# Autodesk Inventor assembly: final
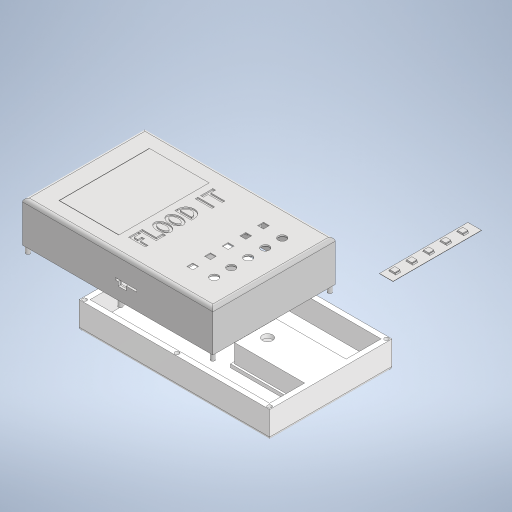
[picture p0: Inventor's stored thumbnail of the model, 512x512]
Saved by Autodesk Inventor 2023 (Build 270158000, 158)
## iProperties
Created: 2022-12-09
Part Number: final
Document SubType Name: Assembly
Designer: spfow
Author: spfow
## Documents named in this file (6)
- C:\Users\spfow\OneDrive\Documents\ECE_414\Final_Project\CAD\final.iam
- C:\Users\spfow\OneDrive\Documents\ECE_414\Final_Project\CAD\Audio_jack.ipt
- C:\Users\spfow\OneDrive\Documents\ECE_414\Final_Project\CAD\CaseBottom.ipt
- C:\Users\spfow\OneDrive\Documents\ECE_414\Final_Project\CAD\CaseTop2.0.ipt
- C:\Users\spfow\OneDrive\Documents\ECE_414\Final_Project\CAD\LCD_Display.ipt
- C:\Users\spfow\OneDrive\Documents\ECE_414\Final_Project\CAD\LED_Strip.ipt
## Components (5 placed, 5 different names)
1. Audio_jack:1 — Mate:3, Mate:4, Mate:5
2. CaseBottom:1
3. CaseTop2.0:1 — Mate:1, Mate:2, Flush:1, Mate:3, Mate:4, Mate:5
4. LCD_Display:1 — Mate:1, Mate:2, Flush:1
5. LED_Strip:1
## Relationships (6: Mate 5, Flush 1)
- Mate:1: CaseTop2.0:1 ↔ LCD_Display:1
- Mate:2: CaseTop2.0:1 ↔ LCD_Display:1
- Flush:1: CaseTop2.0:1 ↔ LCD_Display:1
- Mate:3: Audio_jack:1 ↔ CaseTop2.0:1
- Mate:4: Audio_jack:1 ↔ CaseTop2.0:1
- Mate:5: Audio_jack:1 ↔ CaseTop2.0:1
